# Autodesk Inventor assembly: Tronco
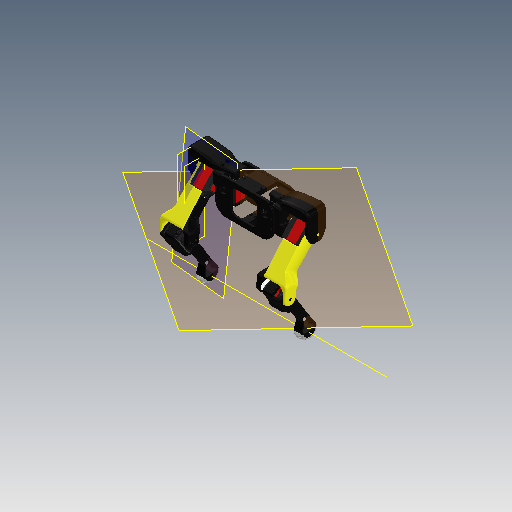
[picture p0: Inventor's stored thumbnail of the model, 512x512]
Saved by Autodesk Inventor 2020 (Build 240168000, 168)
## iProperties
Created: 2022-06-22
Part Number: Tronco
Document SubType Name: Assembly
Designer: JCarlos
Author: JCarlos
## Documents named in this file (4)
- C:\Users\candu\Google Drive\Doutorado_UTFPR\Projeto_1_SpotMicro\Projeto_3D\Robo_Montado_v3\Tronco.iam
- C:\Users\candu\Google Drive\Doutorado_UTFPR\Projeto_1_SpotMicro\Projeto_3D\Robo_Montado_v3\Clavicula.iam
- C:\Users\candu\Google Drive\Doutorado_UTFPR\Projeto_1_SpotMicro\Projeto_3D\Robo_Montado_v3\Perna_Dir_Montada_v3.iam
- C:\Users\candu\Google Drive\Doutorado_UTFPR\Projeto_1_SpotMicro\Projeto_3D\Robo_Montado_v3\Perna_Esq_Montada_v3.iam
## Components (3 placed, 3 different names)
1. Clavicula:1 [sub-assembly] — Coincidência:1, Coincidência:2, Ângulo:1, Ângulo:2, Coincidência:5
2. Perna_Dir_Montada_v3:1 [sub-assembly] — Coincidência:1, Coincidência:2, Coincidência:4, Ângulo:2
3. Perna_Esq_Montada_v3:1 [sub-assembly] — Coincidência:4, Ângulo:1, Coincidência:5
## Relationships (6: Mate 4, Angle 2)
- Coincidência:1 [Mate]: Clavicula:1 ↔ Perna_Dir_Montada_v3:1
- Coincidência:2 [Mate] (2.25 mm): Clavicula:1 ↔ Perna_Dir_Montada_v3:1
- Coincidência:4 [Mate]: Perna_Dir_Montada_v3:1 ↔ Perna_Esq_Montada_v3:1
- Ângulo:1 [Angle] (0 deg): Clavicula:1 ↔ Perna_Esq_Montada_v3:1
- Ângulo:2 [Angle] (0 deg): Clavicula:1 ↔ Perna_Dir_Montada_v3:1
- Coincidência:5 [Mate]: Clavicula:1 ↔ Perna_Esq_Montada_v3:1
